# Autodesk Inventor assembly: Linear Bearing Assembly
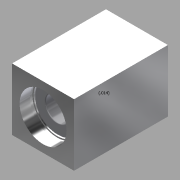
[picture p0: Inventor's stored thumbnail of the model, 180x180]
Saved by Autodesk Inventor 2017 (Build 210142000, 142)
## iProperties
Created: 2017-02-09
Part Number: Linear Bearing Assembly
Document SubType Name: Assembly
Designer: qupec
Author: qupec
## Documents named in this file (3)
- C:\Users\qupec\Desktop\UMD Near Space\RockSat\Linear Bearing Assembly.iam
- C:\Users\qupec\Desktop\UMD Near Space\RockSat\linear bearing.ipt
- C:\Users\qupec\Desktop\UMD Near Space\RockSat\LINEAR SLEEVE BRNG.ipt
## Components (2 placed, 2 different names)
1. linear bearing:1 — Mate:1, Mate:2
2. LINEAR SLEEVE BRNG:1 — Mate:1, Mate:2
## Relationships (2: Mate 2)
- Mate:1: linear bearing:1 ↔ LINEAR SLEEVE BRNG:1
- Mate:2: linear bearing:1 ↔ LINEAR SLEEVE BRNG:1
